# Autodesk Inventor assembly: module_valve
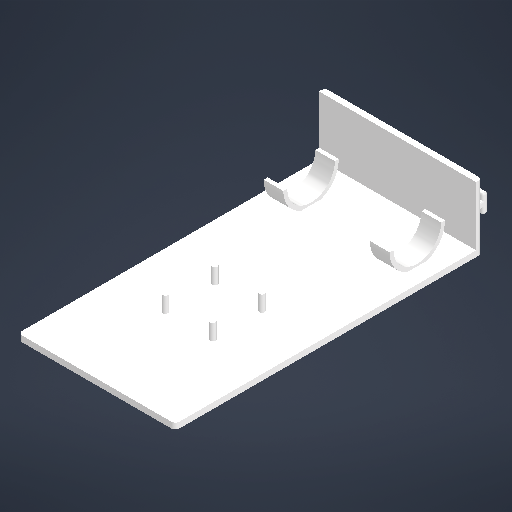
[picture p0: Inventor's stored thumbnail of the model, 512x512]
Saved by Autodesk Inventor 2025.4 (Build 294407000, 407)
## iProperties
Created: 2026-01-03
Part Number: module_valve
Document SubType Name: Assembly
Designer: sam
Author: sam
## Documents named in this file (3)
- G:\projects\primary\regulated-irrigation-system\model\asm\module-valve\module_valve-clips.iam
- G:\projects\primary\regulated-irrigation-system\model\asm\module-valve\module_valve.ipt
- G:\projects\primary\regulated-irrigation-system\model\asm\module-valve\clip-pipe.ipt
## Components (3 placed, 2 different names)
1. module_valve:1 — Mate:4, Mate:5, Mate:6, Mate:7, Mate:8, Mate:9
2. clip-pipe:1 — Mate:7, Mate:8, Mate:9
3. clip-pipe:2 — Mate:4, Mate:5, Mate:6
## Relationships (6: Mate 6)
- Mate:4: module_valve:1 ↔ clip-pipe:2
- Mate:5: module_valve:1 ↔ clip-pipe:2
- Mate:6: module_valve:1 ↔ clip-pipe:2
- Mate:7: module_valve:1 ↔ clip-pipe:1
- Mate:8: module_valve:1 ↔ clip-pipe:1
- Mate:9: module_valve:1 ↔ clip-pipe:1
